# Autodesk Inventor assembly: SP
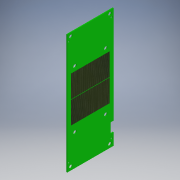
[picture p0: Inventor's stored thumbnail of the model, 180x180]
Saved by Autodesk Inventor 2022 (Build 260153000, 153)
## iProperties
Created: 2021-09-09
Part Number: SP
Document SubType Name: Assembly
Designer: Bowen O'Steen
Author: Bowen O'Steen
## Documents named in this file (3)
- C:\$WorkingFolder\Engineering Data\MemeSat\Solar Panels\SP-01.iam
- C:\$WorkingFolder\Engineering Data\MemeSat\Solar Panels\SolarPCB.ipt
- C:\$WorkingFolder\Engineering Data\MemeSat\Solar Panels\QJcell.ipt
## Components (3 placed, 2 different names)
1. SolarPCB:1 — Mate:1, Mate:2, Flush:1, Mate:3, Mate:4, Angle:1, Angle:2, Mate:5, Flush:2, Flush:3, Mate:6
2. QJcell:1 — Mate:3, Angle:1, Flush:2, Mate:6
3. QJcell:2 — Mate:4, Angle:2, Mate:5, Flush:3
## Relationships (11: Mate 6, Flush 3, Angle 2)
- Mate:1: SolarPCB:1
- Mate:2: SolarPCB:1
- Flush:1: SolarPCB:1
- Mate:3: SolarPCB:1 ↔ QJcell:1
- Mate:4: SolarPCB:1 ↔ QJcell:2
- Angle:1 (0 deg): SolarPCB:1 ↔ QJcell:1
- Angle:2 (0 deg): SolarPCB:1 ↔ QJcell:2
- Mate:5: SolarPCB:1 ↔ QJcell:2
- Flush:2: SolarPCB:1 ↔ QJcell:1
- Flush:3 (3.5 mm): SolarPCB:1 ↔ QJcell:2
- Mate:6 (-2.5 mm): SolarPCB:1 ↔ QJcell:1
